# Autodesk Inventor assembly: S8x1
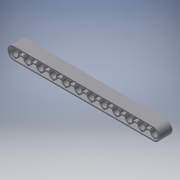
[picture p0: Inventor's stored thumbnail of the model, 180x180]
Saved by Autodesk Inventor 2019 (Build 230136000, 136)
## iProperties
Created: 2019-01-31
Part Number: S8x1
Document SubType Name: Assembly
Designer: Varga Daniel
Author: Varga Daniel
## Documents named in this file (3)
- C:\!_Dani\!_cloud\OneDrive\!_munka\Revolution\RevvyDemoKit\Structural parts\Straight Beams\S12x1.iam
- C:\!_Dani\!_cloud\OneDrive\!_munka\Revolution\RevvyDemoKit\Structural parts\Straight Beams\straight_beam_inner_part_single.ipt
- C:\!_Dani\!_cloud\OneDrive\!_munka\Revolution\RevvyDemoKit\Structural parts\Straight Beams\straight_beam_end_part_single.ipt
## Components (12 placed, 2 different names)
1. straight_beam_inner_part_single:1 — Mate:4, Mate:5, Flush:25, Flush:26, Flush:27, Flush:28, Flush:29, Flush:30
2. straight_beam_inner_part_single:2 — Mate:5, Flush:11, Flush:12, Mate:7, Flush:25, Flush:26
3. straight_beam_inner_part_single:3 — Mate:3, Mate:4, Flush:29, Flush:30
4. straight_beam_inner_part_single:4 — Mate:2, Mate:3, Flush:27, Flush:28, Flush:31, Flush:32
5. straight_beam_inner_part_single:5 — Mate:2, Flush:23, Flush:24, Flush:31, Flush:32, Mate:13
6. straight_beam_end_part_single:1 — Flush:21, Flush:22, Mate:12
7. straight_beam_end_part_single:2 — Flush:11, Flush:12, Mate:7
8. straight_beam_inner_part_single:6 — Flush:13, Flush:14, Mate:8, Flush:15, Flush:16, Mate:9
9. straight_beam_inner_part_single:7 — Flush:15, Flush:16, Mate:9, Flush:17, Flush:18, Mate:10
10. straight_beam_inner_part_single:8 — Flush:17, Flush:18, Mate:10, Flush:19, Flush:20, Mate:11
11. straight_beam_inner_part_single:9 — Flush:19, Flush:20, Mate:11, Flush:21, Flush:22, Mate:12
12. straight_beam_inner_part_single:10 — Flush:13, Flush:14, Mate:8, Flush:23, Flush:24, Mate:13
## Relationships (33: Flush 22, Mate 11)
- Mate:2: straight_beam_inner_part_single:4 ↔ straight_beam_inner_part_single:5
- Mate:3: straight_beam_inner_part_single:3 ↔ straight_beam_inner_part_single:4
- Mate:4: straight_beam_inner_part_single:1 ↔ straight_beam_inner_part_single:3
- Mate:5: straight_beam_inner_part_single:1 ↔ straight_beam_inner_part_single:2
- Flush:11: straight_beam_inner_part_single:2 ↔ straight_beam_end_part_single:2
- Flush:12: straight_beam_inner_part_single:2 ↔ straight_beam_end_part_single:2
- Mate:7: straight_beam_inner_part_single:2 ↔ straight_beam_end_part_single:2
- Flush:13: straight_beam_inner_part_single:6 ↔ straight_beam_inner_part_single:10
- Flush:14: straight_beam_inner_part_single:6 ↔ straight_beam_inner_part_single:10
- Mate:8: straight_beam_inner_part_single:6 ↔ straight_beam_inner_part_single:10
- Flush:15: straight_beam_inner_part_single:6 ↔ straight_beam_inner_part_single:7
- Flush:16: straight_beam_inner_part_single:6 ↔ straight_beam_inner_part_single:7
- Mate:9: straight_beam_inner_part_single:6 ↔ straight_beam_inner_part_single:7
- Flush:17: straight_beam_inner_part_single:7 ↔ straight_beam_inner_part_single:8
- Flush:18: straight_beam_inner_part_single:7 ↔ straight_beam_inner_part_single:8
- Mate:10: straight_beam_inner_part_single:7 ↔ straight_beam_inner_part_single:8
- Flush:19: straight_beam_inner_part_single:8 ↔ straight_beam_inner_part_single:9
- Flush:20: straight_beam_inner_part_single:8 ↔ straight_beam_inner_part_single:9
- Mate:11: straight_beam_inner_part_single:8 ↔ straight_beam_inner_part_single:9
- Flush:21: straight_beam_end_part_single:1 ↔ straight_beam_inner_part_single:9
- Flush:22: straight_beam_end_part_single:1 ↔ straight_beam_inner_part_single:9
- Mate:12: straight_beam_end_part_single:1 ↔ straight_beam_inner_part_single:9
- Flush:23: straight_beam_inner_part_single:5 ↔ straight_beam_inner_part_single:10
- Flush:24: straight_beam_inner_part_single:5 ↔ straight_beam_inner_part_single:10
- Flush:25: straight_beam_inner_part_single:1 ↔ straight_beam_inner_part_single:2
- Flush:26: straight_beam_inner_part_single:1 ↔ straight_beam_inner_part_single:2
- Flush:27: straight_beam_inner_part_single:1 ↔ straight_beam_inner_part_single:4
- Flush:28: straight_beam_inner_part_single:1 ↔ straight_beam_inner_part_single:4
- Flush:29: straight_beam_inner_part_single:1 ↔ straight_beam_inner_part_single:3
- Flush:30: straight_beam_inner_part_single:1 ↔ straight_beam_inner_part_single:3
- Flush:31: straight_beam_inner_part_single:4 ↔ straight_beam_inner_part_single:5
- Flush:32: straight_beam_inner_part_single:4 ↔ straight_beam_inner_part_single:5
- Mate:13: straight_beam_inner_part_single:5 ↔ straight_beam_inner_part_single:10
